# Autodesk Inventor assembly: Base Assembly
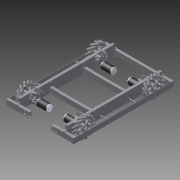
[picture p0: Inventor's stored thumbnail of the model, 180x180]
Saved by Autodesk Inventor 2015 (Build 190159000, 159)
## iProperties
Created: 2015-01-14
Part Number: Base Assembly
Document SubType Name: Assembly
Designer: chapale16
Author: chapale16
## Documents named in this file (29)
- \\lhssvr02\Homedirs\Robotics Club\CAD Model 2015\CDR prep\Frame\Base Assembly.iam
- \\lhssvr02\Homedirs\Robotics Club\CAD Model 2015\CDR prep\Frame\Frame front-back.ipt
- \\lhssvr02\Homedirs\Robotics Club\CAD Model 2015\Parts Folder\Wheels\Right Vex Mec Wheel_MIR.iam
- \\lhssvr02\Homedirs\Robotics Club\CAD Model 2015\2x1 boxbeam 18 in.ipt
- \\lhssvr02\Homedirs\Robotics Club\CAD Model 2015\CDR prep\Frame\Standoffs Large_MIR.ipt
- \\lhssvr02\Homedirs\Robotics Club\CAD Model 2015\L-Gusset.ipt
- \\lhssvr02\Homedirs\Robotics Club\CAD Model 2015\CDR prep\Frame\bumper piece.ipt
- \\lhssvr02\Homedirs\Robotics Club\CAD Model 2015\Modified Front Frame 27 in_MIR_MIR1.ipt
- \\lhssvr02\Homedirs\Robotics Club\CAD Model 2015\CDR prep\Frame\Standoffs Large_MIR_MIR.ipt
- \\lhssvr02\Homedirs\Robotics Club\CAD Model 2015\L-Gusset_MIR.ipt
- \\lhssvr02\Homedirs\Robotics Club\CAD Model 2015\CDR prep\Frame\boxbeam 4x1 with sideways holes_MIR.ipt
- \\lhssvr02\Homedirs\Robotics Club\CAD Model 2015\Parts Folder\Motors\Imported Components\MOT_CIM-Motor_217-2000.iam\FR801-001_CIM Motor Body_MIR2.ipt
- \\lhssvr02\Homedirs\Robotics Club\CAD Model 2015\Box Beam Drive Base\Newest\Toughbox-mini (1)_MIR2.iam
- \\lhssvr02\Homedirs\Robotics Club\CAD Model 2015\Box Beam Drive Base\Newest\3x5 T.ipt
- \\lhssvr02\Homedirs\Robotics Club\CAD Model 2015\Box Beam Drive Base\Newest\3x5 T_MIR1.ipt
- \\lhssvr02\Homedirs\Robotics Club\CAD Model 2015\Box Beam Drive Base\Newest\3x5 T_MIR2.ipt
- \\lhssvr02\Homedirs\Robotics Club\CAD Model 2015\Box Beam Drive Base\Newest\3x5 T_MIR1_MIR.ipt
- \\lhssvr02\Homedirs\Robotics Club\CAD Model 2015\Modified Front Frame 27 in_MIR_MIR1_MIR.ipt
- \\lhssvr02\Homedirs\Robotics Club\CAD Model 2015\Box Beam Drive Base\34Assembly.ipt
- \\lhssvr02\Homedirs\Robotics Club\CAD Model 2015\CDR prep\Frame\Standoffs Large_MIR_MIR_MIR.ipt
- \\lhssvr02\Homedirs\Robotics Club\CAD Model 2015\Parts Folder\Wheels\Right Vex Mec Wheel_MIR_MIR1.iam
- \\lhssvr02\Homedirs\Robotics Club\CAD Model 2015\Parts Folder\Motors\Imported Components\MOT_CIM-Motor_217-2000.iam\FR801-001_CIM Motor Body_MIR2_MIR.ipt
- \\lhssvr02\Homedirs\Robotics Club\CAD Model 2015\Box Beam Drive Base\Newest\Toughbox-mini (1)_MIR2_MIR.iam
- \\lhssvr02\Homedirs\Robotics Club\CAD Model 2015\Parts Folder\Wheels\Right Vex Mec Wheel_MIR_MIR2.iam
- \\lhssvr02\Homedirs\Robotics Club\CAD Model 2015\Parts Folder\Motors\Imported Components\MOT_CIM-Motor_217-2000.iam\FR801-001_CIM Motor Body_MIR2_MIR1.ipt
- \\lhssvr02\Homedirs\Robotics Club\CAD Model 2015\Box Beam Drive Base\Newest\Toughbox-mini (1)_MIR2_MIR1.iam
- \\lhssvr02\Homedirs\Robotics Club\CAD Model 2015\Parts Folder\Wheels\Right Vex Mec Wheel_MIR_MIR1_MIR.iam
- \\lhssvr02\Homedirs\Robotics Club\CAD Model 2015\Parts Folder\Motors\Imported Components\MOT_CIM-Motor_217-2000.iam\FR801-001_CIM Motor Body_MIR2_MIR_MIR.ipt
- \\lhssvr02\Homedirs\Robotics Club\CAD Model 2015\Box Beam Drive Base\Newest\Toughbox-mini (1)_MIR2_MIR_MIR.iam
## Components (43 placed, 28 different names)
1. Frame front-back:2 — Flush:60, Mate:121, Tangent:3, Mate:123, Tangent:4
2. Right Vex Mec Wheel_MIR:1 [sub-assembly] — Mate:104
3. 2x1 boxbeam 18 in:1 — Mate:64, Flush:34, Mate:66, Flush:35, Flush:66
4. Standoffs Large_MIR:1
5. Standoffs Large_MIR:2
6. 2x1 boxbeam 18 in:2 — Mate:62, Flush:33, Mate:69, Flush:36, Flush:68
7. L-Gusset:1 — Mate:62, Flush:33
8. L-Gusset:2 — Mate:64, Flush:34, Mate:115
9. L-Gusset:3 — Mate:69, Flush:36
10. L-Gusset:4 — Mate:66, Flush:35
11. Modified Front Frame 27 in_MIR_MIR1:1 — Mate:93, Flush:59, Flush:63, Mate:112, Mate:116, Tangent:2
12. Standoffs Large_MIR_MIR:1 — Mate:124, Mate:125
13. L-Gusset_MIR:1
14. L-Gusset_MIR:2 — Mate:94
15. boxbeam 4x1 with sideways holes_MIR:1 — Mate:93, Mate:94, Flush:59, Flush:64, Flush:65, Mate:113, Flush:67, Mate:117, Mate:120
16. FR801-001_CIM Motor Body_MIR2:1 — Mate:100, Tangent:8
17. Toughbox-mini (1)_MIR2:1 [sub-assembly] — Mate:100, Mate:104, Mate:131, Mate:132, Mate:135, Tangent:8
18. bumper piece:1
19. bumper piece:2 — Mate:124, Mate:125
20. 3x5 T:1 — Flush:63, Mate:112, Flush:64
21. 3x5 T:2 — Flush:65, Mate:113, Flush:66
22. 3x5 T:3 — Flush:67, Flush:68
23. 3x5 T_MIR1:1
24. 3x5 T_MIR2:1
25. 3x5 T_MIR2:2 — Mate:114
26. 3x5 T_MIR2:3
27. 3x5 T_MIR1_MIR:1
28. boxbeam 4x1 with sideways holes_MIR:2 — Mate:114, Mate:115, Mate:118, Mate:122, Mate:129, Mate:130, Mate:135
29. Modified Front Frame 27 in_MIR_MIR1_MIR:1 — Mate:119, Tangent:1
30. 34Assembly:1 — Mate:116, Mate:117, Tangent:2
31. 34Assembly:2 — Mate:118, Mate:119, Tangent:1
32. 34Assembly:3 — Mate:120, Mate:121, Tangent:3
33. 34Assembly:4 — Mate:122, Mate:123, Tangent:4
34. Standoffs Large_MIR_MIR_MIR:1
35. Right Vex Mec Wheel_MIR_MIR1:1 [sub-assembly] — Mate:136
36. FR801-001_CIM Motor Body_MIR2_MIR:1 — Mate:138, Tangent:7
37. Toughbox-mini (1)_MIR2_MIR:1 [sub-assembly] — Mate:136, Mate:138, Mate:139, Mate:140, Tangent:7
38. Right Vex Mec Wheel_MIR_MIR2:1 [sub-assembly] — Mate:141
39. FR801-001_CIM Motor Body_MIR2_MIR1:1 — Mate:143, Tangent:5
40. Toughbox-mini (1)_MIR2_MIR1:1 [sub-assembly] — Mate:141, Mate:143, Mate:144, Mate:145, Tangent:5
41. Right Vex Mec Wheel_MIR_MIR1_MIR:1 [sub-assembly] — Mate:148
42. FR801-001_CIM Motor Body_MIR2_MIR_MIR:1 — Mate:146, Tangent:6
43. Toughbox-mini (1)_MIR2_MIR_MIR:1 [sub-assembly] — Mate:146, Mate:148, Mate:149, Mate:150, Tangent:6
## Relationships (61: Mate 41, Flush 12, Tangent 8)
- Mate:62: 2x1 boxbeam 18 in:2 ↔ L-Gusset:1
- Flush:33: 2x1 boxbeam 18 in:2 ↔ L-Gusset:1
- Mate:64: 2x1 boxbeam 18 in:1 ↔ L-Gusset:2
- Flush:34: 2x1 boxbeam 18 in:1 ↔ L-Gusset:2
- Mate:66: 2x1 boxbeam 18 in:1 ↔ L-Gusset:4
- Flush:35: 2x1 boxbeam 18 in:1 ↔ L-Gusset:4
- Mate:69: 2x1 boxbeam 18 in:2 ↔ L-Gusset:3
- Flush:36: 2x1 boxbeam 18 in:2 ↔ L-Gusset:3
- Mate:93: Modified Front Frame 27 in_MIR_MIR1:1 ↔ boxbeam 4x1 with sideways holes_MIR:1
- Mate:94: L-Gusset_MIR:2 ↔ boxbeam 4x1 with sideways holes_MIR:1
- Flush:59: Modified Front Frame 27 in_MIR_MIR1:1 ↔ boxbeam 4x1 with sideways holes_MIR:1
- Flush:60 (482.6 mm): Frame front-back:2
- Mate:100: FR801-001_CIM Motor Body_MIR2:1 ↔ Toughbox-mini (1)_MIR2:1
- Mate:104: Right Vex Mec Wheel_MIR:1 ↔ Toughbox-mini (1)_MIR2:1
- Flush:63 (1.5875 mm): Modified Front Frame 27 in_MIR_MIR1:1 ↔ 3x5 T:1
- Mate:112: Modified Front Frame 27 in_MIR_MIR1:1 ↔ 3x5 T:1
- Flush:64 (1.5875 mm): boxbeam 4x1 with sideways holes_MIR:1 ↔ 3x5 T:1
- Flush:65 (1.5875 mm): boxbeam 4x1 with sideways holes_MIR:1 ↔ 3x5 T:2
- Mate:113: boxbeam 4x1 with sideways holes_MIR:1 ↔ 3x5 T:2
- Flush:66 (1.5875 mm): 2x1 boxbeam 18 in:1 ↔ 3x5 T:2
- Flush:67 (1.5875 mm): boxbeam 4x1 with sideways holes_MIR:1 ↔ 3x5 T:3
- Flush:68 (1.5875 mm): 2x1 boxbeam 18 in:2 ↔ 3x5 T:3
- Mate:114: 3x5 T_MIR2:2 ↔ boxbeam 4x1 with sideways holes_MIR:2
- Mate:115: L-Gusset:2 ↔ boxbeam 4x1 with sideways holes_MIR:2
- Mate:116: Modified Front Frame 27 in_MIR_MIR1:1 ↔ 34Assembly:1
- Mate:117: boxbeam 4x1 with sideways holes_MIR:1 ↔ 34Assembly:1
- Mate:118: boxbeam 4x1 with sideways holes_MIR:2 ↔ 34Assembly:2
- Mate:119: Modified Front Frame 27 in_MIR_MIR1_MIR:1 ↔ 34Assembly:2
- Tangent:1: Modified Front Frame 27 in_MIR_MIR1_MIR:1 ↔ 34Assembly:2
- Tangent:2: Modified Front Frame 27 in_MIR_MIR1:1 ↔ 34Assembly:1
- Mate:120: boxbeam 4x1 with sideways holes_MIR:1 ↔ 34Assembly:3
- Mate:121: Frame front-back:2 ↔ 34Assembly:3
- Tangent:3: Frame front-back:2 ↔ 34Assembly:3
- Mate:122: boxbeam 4x1 with sideways holes_MIR:2 ↔ 34Assembly:4
- Mate:123: Frame front-back:2 ↔ 34Assembly:4
- Tangent:4: Frame front-back:2 ↔ 34Assembly:4
- Mate:124 (-25.4 mm): Standoffs Large_MIR_MIR:1 ↔ bumper piece:2
- Mate:125: Standoffs Large_MIR_MIR:1 ↔ bumper piece:2
- Mate:129: boxbeam 4x1 with sideways holes_MIR:2
- Mate:130: boxbeam 4x1 with sideways holes_MIR:2
- Mate:131: Toughbox-mini (1)_MIR2:1
- Mate:132: Toughbox-mini (1)_MIR2:1
- Mate:133
- Mate:134
- Mate:135: Toughbox-mini (1)_MIR2:1 ↔ boxbeam 4x1 with sideways holes_MIR:2
- Mate:136: Right Vex Mec Wheel_MIR_MIR1:1 ↔ Toughbox-mini (1)_MIR2_MIR:1
- Mate:138: FR801-001_CIM Motor Body_MIR2_MIR:1 ↔ Toughbox-mini (1)_MIR2_MIR:1
- Mate:139: Toughbox-mini (1)_MIR2_MIR:1
- Mate:140: Toughbox-mini (1)_MIR2_MIR:1
- Mate:141: Right Vex Mec Wheel_MIR_MIR2:1 ↔ Toughbox-mini (1)_MIR2_MIR1:1
- Mate:143: FR801-001_CIM Motor Body_MIR2_MIR1:1 ↔ Toughbox-mini (1)_MIR2_MIR1:1
- Mate:144: Toughbox-mini (1)_MIR2_MIR1:1
- Mate:145: Toughbox-mini (1)_MIR2_MIR1:1
- Mate:146: FR801-001_CIM Motor Body_MIR2_MIR_MIR:1 ↔ Toughbox-mini (1)_MIR2_MIR_MIR:1
- Mate:148: Right Vex Mec Wheel_MIR_MIR1_MIR:1 ↔ Toughbox-mini (1)_MIR2_MIR_MIR:1
- Mate:149: Toughbox-mini (1)_MIR2_MIR_MIR:1
- Mate:150: Toughbox-mini (1)_MIR2_MIR_MIR:1
- Tangent:5: FR801-001_CIM Motor Body_MIR2_MIR1:1 ↔ Toughbox-mini (1)_MIR2_MIR1:1
- Tangent:6: FR801-001_CIM Motor Body_MIR2_MIR_MIR:1 ↔ Toughbox-mini (1)_MIR2_MIR_MIR:1
- Tangent:7: FR801-001_CIM Motor Body_MIR2_MIR:1 ↔ Toughbox-mini (1)_MIR2_MIR:1
- Tangent:8: FR801-001_CIM Motor Body_MIR2:1 ↔ Toughbox-mini (1)_MIR2:1
